# Autodesk Inventor assembly: Mount
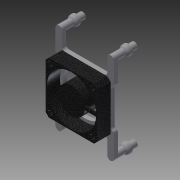
[picture p0: Inventor's stored thumbnail of the model, 180x180]
Saved by Autodesk Inventor 2013 (Build 170138000, 138)
## iProperties
Created: 2014-11-16
Part Number: Mount
Document SubType Name: Assembly
Designer: Kyle
Author: Kyle
## Documents named in this file (3)
- C:\Users\Kyle\Documents\Autodesk\Output\Inventor 2013\Motor Driver Fan Mount V1.2\Mount.iam
- C:\Users\Kyle\Documents\Autodesk\Output\Inventor 2013\Motor Driver Fan Mount V1.2\Base.ipt
- C:\Users\Kyle\Documents\Autodesk\Output\Inventor 2013\Motor Driver Fan Mount V1.2\Fan.ipt
## Components (2 placed, 2 different names)
1. Base:1 — Mate:3, Mate:11, Mate:12
2. Fan:1 — Mate:3, Mate:11, Mate:12
## Relationships (3: Mate 3)
- Mate:3: Base:1 ↔ Fan:1
- Mate:11: Base:1 ↔ Fan:1
- Mate:12: Base:1 ↔ Fan:1
